# Autodesk Inventor assembly: Assy_cam_connection
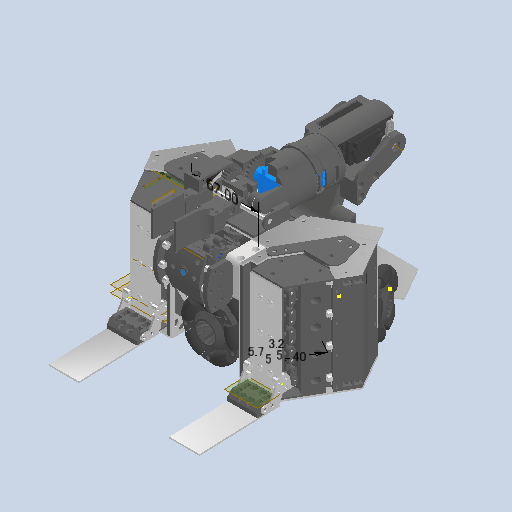
[picture p0: Inventor's stored thumbnail of the model, 512x512]
Saved by Autodesk Inventor 2024.1 (Build 281209000, 209)
## iProperties
Created: 2025-03-04
Part Number: Assy_cam_connection
Document SubType Name: Assembly
Designer: hibik
Author: hibik
## Documents named in this file (8)
- C:\Users\hibik\Documents\Robomech\RESCUE\ORCA\hard\Assy_cam_connection.iam
- C:\Users\hibik\Documents\Robomech\RESCUE\ORCA\hard\Assy_fork_connection.iam
- C:\Users\hibik\Documents\Robomech\RESCUE\ORCA\hard\camera\cam_set.iam
- C:\Users\hibik\Documents\Robomech\RESCUE\ORCA\hard\flame_front\cam_setter_right_under.ipt
- C:\Users\hibik\Documents\Robomech\RESCUE\ORCA\hard\flame_front\cam_setter_right_upper.ipt
- C:\Users\hibik\Documents\Robomech\RESCUE\ORCA\hard\flame_front\cam_setter_left_under.ipt
- C:\Users\hibik\Documents\Robomech\RESCUE\ORCA\hard\flame_front\cam_setter_left_upper.ipt
- C:\Users\hibik\Documents\Robomech\RESCUE\ORCA\hard\arm\Assy_arm.iam
## Components (7 placed, 7 different names)
1. Assy_fork_connection:1 [sub-assembly] — 挿入:1, 挿入:2, 角度:1, メイト:2, 挿入:4, 挿入:5, 挿入:8, 挿入:9
2. cam_set:1 [sub-assembly] — 挿入:3, 角度:1
3. cam_setter_right_under:1 — 挿入:1, 挿入:2, 挿入:3, フラッシュ:1, メイト:1
4. cam_setter_right_upper:1 — フラッシュ:1, メイト:1, メイト:2
5. cam_setter_left_under:1 — 挿入:4, 挿入:5, 挿入:6, 挿入:7
6. cam_setter_left_upper:1 — 挿入:6, 挿入:7
7. Assy_arm:1 [sub-assembly] — 挿入:8, 挿入:9
## Relationships (13: Insert 9, Mate 2, Angle 1, Flush 1)
- 挿入:1 [Insert]: Assy_fork_connection:1 ↔ cam_setter_right_under:1
- 挿入:2 [Insert]: Assy_fork_connection:1 ↔ cam_setter_right_under:1
- 挿入:3 [Insert]: cam_set:1 ↔ cam_setter_right_under:1
- 角度:1 [Angle] (0 deg): Assy_fork_connection:1 ↔ cam_set:1
- フラッシュ:1 [Flush]: cam_setter_right_under:1 ↔ cam_setter_right_upper:1
- メイト:1 [Mate]: cam_setter_right_under:1 ↔ cam_setter_right_upper:1
- メイト:2 [Mate]: Assy_fork_connection:1 ↔ cam_setter_right_upper:1
- 挿入:4 [Insert]: Assy_fork_connection:1 ↔ cam_setter_left_under:1
- 挿入:5 [Insert]: Assy_fork_connection:1 ↔ cam_setter_left_under:1
- 挿入:6 [Insert]: cam_setter_left_under:1 ↔ cam_setter_left_upper:1
- 挿入:7 [Insert]: cam_setter_left_under:1 ↔ cam_setter_left_upper:1
- 挿入:8 [Insert]: Assy_fork_connection:1 ↔ Assy_arm:1
- 挿入:9 [Insert]: Assy_fork_connection:1 ↔ Assy_arm:1
